# Autodesk Inventor assembly: Panto_Latch_Leg
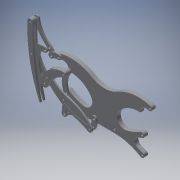
[picture p0: Inventor's stored thumbnail of the model, 180x180]
Saved by Autodesk Inventor 2017 (Build 210142000, 142)
## iProperties
Created: 2016-08-27
Part Number: Panto_Latch_Leg
Document SubType Name: Assembly
Designer: Nic
Author: Nic
## Documents named in this file (11)
- C:\Users\Nic\Documents\TermiteBeest\Panto_Latch_Leg.iam
- C:\Users\Nic\Documents\TermiteBeest\legB.ipt
- C:\Users\Nic\Documents\TermiteBeest\legFrame_Panto.ipt
- C:\Users\Nic\Documents\TermiteBeest\linkageC_mini.ipt
- C:\Users\Nic\Documents\TermiteBeest\linkageB_mini.ipt
- C:\Users\Nic\Documents\TermiteBeest\linkageA_mini.ipt
- C:\Users\Nic\Documents\TermiteBeest\legA_mini.ipt
- C:\Users\Nic\Documents\TermiteBeest\panto_linkagedi.ipt
- C:\Users\Nic\Documents\TermiteBeest\panto_linkageE.ipt
- C:\Users\Nic\Documents\TermiteBeest\panto_legA.ipt
- C:\Users\Nic\Documents\TermiteBeest\panto_linkageF.ipt
## Components (12 placed, 10 different names)
1. legB:1 — Insert:4, Insert:5, Insert:9, Insert:20
2. legFrame_Panto:1 — Insert:1, Insert:2, Insert:3, Insert:8, Insert:10
3. linkageC_mini:1 — Insert:1, Insert:5
4. linkageB_mini:1 — Insert:2, Insert:4
5. linkageA_mini:1 — Insert:3, Insert:19
6. legA_mini:1 — Insert:17, Insert:18, Insert:19, Insert:20
7. linkageC_mini:2 — Insert:8, Insert:9
8. linkageC_mini:3 — Insert:10, Insert:11
9. panto_linkagedi:1 — Insert:11, Insert:13, Insert:16
10. panto_linkageE:1 — Insert:15, Insert:18
11. panto_legA:1 — Insert:13, Insert:15
12. panto_linkageF:1 — Insert:16, Insert:17
## Relationships (16: Insert 16)
- Insert:1: legFrame_Panto:1 ↔ linkageC_mini:1
- Insert:2 (2 mm): legFrame_Panto:1 ↔ linkageB_mini:1
- Insert:3: legFrame_Panto:1 ↔ linkageA_mini:1
- Insert:4: legB:1 ↔ linkageB_mini:1
- Insert:5 (2 mm): legB:1 ↔ linkageC_mini:1
- Insert:8: legFrame_Panto:1 ↔ linkageC_mini:2
- Insert:9 (2 mm): legB:1 ↔ linkageC_mini:2
- Insert:10: legFrame_Panto:1 ↔ linkageC_mini:3
- Insert:11: linkageC_mini:3 ↔ panto_linkagedi:1
- Insert:13 (1.5 mm): panto_linkagedi:1 ↔ panto_legA:1
- Insert:15: panto_linkageE:1 ↔ panto_legA:1
- Insert:16 (3 mm): panto_linkagedi:1 ↔ panto_linkageF:1
- Insert:17: legA_mini:1 ↔ panto_linkageF:1
- Insert:18: legA_mini:1 ↔ panto_linkageE:1
- Insert:19: linkageA_mini:1 ↔ legA_mini:1
- Insert:20 (0.5 mm): legB:1 ↔ legA_mini:1
